# Autodesk Inventor assembly: RisingCam-Takumar
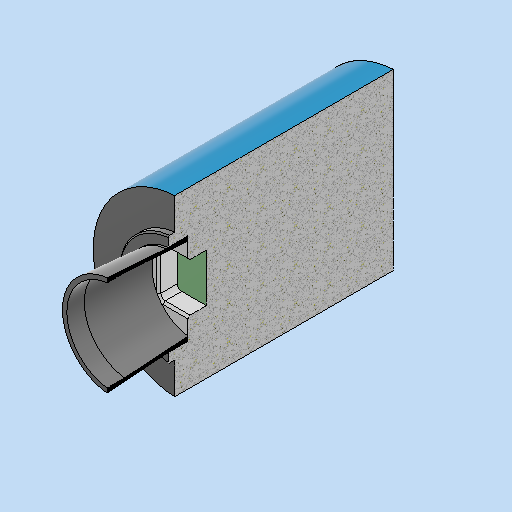
[picture p0: Inventor's stored thumbnail of the model, 512x512]
Saved by Autodesk Inventor 2025 (Build 290162000, 162)
## iProperties
Created: 2025-02-21
Part Number: RisingCam-Takumar
Document SubType Name: Assembly
Designer: kuzmin
Author: kuzmin
## Documents named in this file (3)
- C:\Users\queez\Dropbox\Drawings\PIHTI\Jobin-Yvon\RisingCam-Takumar.iam
- C:\Users\queez\Dropbox\Drawings\PIHTI\Jobin-Yvon\RisingCam-IMX571.ipt
- C:\Users\queez\Dropbox\Drawings\PIHTI\Jobin-Yvon\Takumar-to-RisingCam.ipt
## Components (2 placed, 2 different names)
1. RisingCam-IMX571:1 — Mate:1, Flush:1
2. Takumar-to-RisingCam:1 — Mate:1, Flush:1
## Relationships (2: Mate 1, Flush 1)
- Mate:1: RisingCam-IMX571:1 ↔ Takumar-to-RisingCam:1
- Flush:1 (-45.5 mm): RisingCam-IMX571:1 ↔ Takumar-to-RisingCam:1
